# Autodesk Inventor assembly: airhockeybot_table_simulation_centered
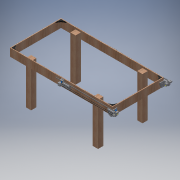
[picture p0: Inventor's stored thumbnail of the model, 180x180]
Saved by Autodesk Inventor 2019.3 (Build 233278000, 278)
## iProperties
Created: 2020-12-03
Part Number: airhockeybot_table_simulation_centered
Material: Generisch
Document SubType Name: Assembly
Designer: Nicolas Frick
Author: Nicolas Frick
## Documents named in this file (2)
- C:\Users\Nicolas Frick\Sync\OneDrive\airhockeybot\mechanical_design\inventor\airhockeybot_table_simulation_centered.iam
- C:\Users\Nicolas Frick\Sync\OneDrive\airhockeybot\mechanical_design\inventor\airhockeybot_table_simulation.iam
## Components (1 placed, 1 different names)
1. airhockeybot_table_simulation:1 [sub-assembly] — Passend:1, Passend:2, Passend:3
## Relationships (3: Mate 3)
- Passend:1 [Mate]: airhockeybot_table_simulation:1
- Passend:2 [Mate]: airhockeybot_table_simulation:1
- Passend:3 [Mate]: airhockeybot_table_simulation:1
